# Autodesk Inventor assembly: 2AM-17-A-0200 - slider motor and gearbox
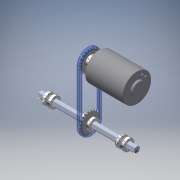
[picture p0: Inventor's stored thumbnail of the model, 180x180]
Saved by Autodesk Inventor 2017 (Build 210142000, 142)
## iProperties
Created: 2017-12-28
Part Number: 2AM-17-A-0200 - slider motor and gearbox
Document SubType Name: Assembly
Designer: Micah
Author: Micah
## Documents named in this file (8)
- C:\Users\Micah\Desktop\inventor\CADathon-2017\2AM-17-A-0200 - Smokestack Elevator\2AM-17-A-7200 - slider motor and gearbox.iam
- C:\Users\Micah\Desktop\inventor\COTS\Motors\Mini CIM Motor\217-3371-STEP.ipt
- C:\Users\Micah\Desktop\inventor\CADathon-2017\2AM-17-A-0200 - Smokestack Elevator\COTS\217-2761-STEP.ipt
- C:\Users\Micah\Desktop\inventor\CADathon-2017\2AM-17-A-0200 - Smokestack Elevator\COTS\217-3255-STEP.ipt
- C:\Users\Micah\Desktop\inventor\CADathon-2017\2AM-17-A-0200 - Smokestack Elevator\COTS\217-2737.20121205.ipt
- C:\Users\Micah\Desktop\inventor\CADathon-2017\2AM-17-A-0200 - Smokestack Elevator\2AM-17-P-7201 - sproket thing ig.ipt
- C:\Users\Micah\Desktop\inventor\CADathon-2017\2AM-17-A-0200 - Smokestack Elevator\2AM-17-A-7200 - slider motor and gearbox\Design Accelerator\Chain Drive2.iam
- C:\Users\Micah\Desktop\inventor\CADathon-2017\2AM-17-A-0200 - Smokestack Elevator\2AM-17-P-7202 - hex shaft.ipt
## Components (16 placed, 7 different names)
1. 217-3371-STEP:1 — Mate:1, Insert:1, Rotational:2, Rotational:3, Rotational:4
2. 217-2761-STEP:2 — Mate:1
3. 217-3255-STEP:1 — Insert:1
4. 217-2737.20121205:1 — Rotational:2
5. 217-2737.20121205:2 — Rotational:3
6. 2AM-17-P-7201 - sproket thing ig:1 — Rotational:4
7. Chain Drive:1 [sub-assembly] — Rotational:5
8. 2AM-17-P-7202 - hex shaft:1 — Rotational:5, Rigid:1, Rigid:2, Rigid:3, Rigid:4, Rigid:5, Rigid:6, Rigid:7, Rigid:8
9. 2AM-17-P-7201 - sproket thing ig:2 — Rigid:2
10. 2AM-17-P-7201 - sproket thing ig:3 — Rigid:1
11. 217-2737.20121205:3 — Rigid:3
12. 217-2737.20121205:4 — Rigid:4
13. 217-2737.20121205:5 — Rigid:6
14. 217-2737.20121205:6 — Rigid:8
15. 217-2737.20121205:7 — Rigid:7
16. 217-2737.20121205:8 — Rigid:5
## Relationships (14: WeldJoint 8, RevoluteJoint 4, Mate 1, Insert 1)
- Mate:1: 217-3371-STEP:1 ↔ 217-2761-STEP:2
- Insert:1 (-28.575 mm): 217-3371-STEP:1 ↔ 217-3255-STEP:1
- Rotational:2 [RevoluteJoint] (-11.43 mm): 217-3371-STEP:1 ↔ 217-2737.20121205:1
- Rotational:3 [RevoluteJoint] (-16.51 mm): 217-3371-STEP:1 ↔ 217-2737.20121205:2
- Rotational:4 [RevoluteJoint] (-15.24 mm): 217-3371-STEP:1 ↔ 2AM-17-P-7201 - sproket thing ig:1
- Rotational:5 [RevoluteJoint] (-107.95 mm): Chain Drive:1 ↔ 2AM-17-P-7202 - hex shaft:1
- Rigid:1 [WeldJoint] (-25.4 mm): 2AM-17-P-7202 - hex shaft:1 ↔ 2AM-17-P-7201 - sproket thing ig:3
- Rigid:2 [WeldJoint] (-25.4 mm): 2AM-17-P-7202 - hex shaft:1 ↔ 2AM-17-P-7201 - sproket thing ig:2
- Rigid:3 [WeldJoint] (-33.02 mm): 2AM-17-P-7202 - hex shaft:1 ↔ 217-2737.20121205:3
- Rigid:4 [WeldJoint] (-14.2875 mm): 2AM-17-P-7202 - hex shaft:1 ↔ 217-2737.20121205:4
- Rigid:5 [WeldJoint] (-98.425 mm): 2AM-17-P-7202 - hex shaft:1 ↔ 217-2737.20121205:8
- Rigid:6 [WeldJoint] (-36.5125 mm): 2AM-17-P-7202 - hex shaft:1 ↔ 217-2737.20121205:5
- Rigid:7 [WeldJoint] (-23.8125 mm): 2AM-17-P-7202 - hex shaft:1 ↔ 217-2737.20121205:7
- Rigid:8 [WeldJoint] (-101.6 mm): 2AM-17-P-7202 - hex shaft:1 ↔ 217-2737.20121205:6
